# Autodesk Inventor assembly: Лестница
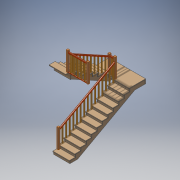
[picture p0: Inventor's stored thumbnail of the model, 180x180]
Saved by Autodesk Inventor 2019 (Build 230136000, 136)
## iProperties
Created: 2018-10-10
Part Number: Лестница
Material: Типовые
Document SubType Name: Assembly
Designer: Андреев Н.Л.
Mass: 392363 g
Surface Area: 432794 cm^2
Volume: 616684 cm^3
Density: 0.636246 g/cm^3
_SolveAssemblyDoc: Frame Generator Solve Assembly
_Version: 15.0.0
Author: Андреев Н.Л.
## Documents named in this file (15)
- C:\Users\andrnl\Documents\Inventor\Мурзин\Лестница.iam
- C:\Users\andrnl\Documents\Inventor\Мурзин\Проступь\Проступь-02.ipt
- C:\Users\andrnl\Documents\Inventor\Мурзин\Проступь.ipt
- C:\Users\andrnl\Documents\Inventor\Мурзин\Марш\Марш-01.iam
- C:\Users\andrnl\Documents\Inventor\Мурзин\Марш.iam
- C:\Users\andrnl\Documents\Inventor\Мурзин\Марш\Марш-02.iam
- C:\Users\andrnl\Documents\Inventor\Мурзин\Столб\Столб-01.ipt
- C:\Users\andrnl\Documents\Inventor\Мурзин\Столб.ipt
- C:\Users\andrnl\Documents\Inventor\Мурзин\Лестница\Frame\Frame0001.iam
- C:\Users\andrnl\Documents\Inventor\Мурзин\Балясина\Балясина-01.ipt
- C:\Users\andrnl\Documents\Inventor\Мурзин\Балясина.ipt
- C:\Users\andrnl\Documents\Inventor\Мурзин\Балясина\Балясина-02.ipt
- C:\Users\andrnl\Documents\Inventor\Мурзин\Проступь\Проступь-01.ipt
- C:\Users\andrnl\Documents\Inventor\Мурзин\Балка.ipt
- C:\Users\andrnl\Documents\Inventor\Мурзин\Лестница Мурзин.xlsx
## Components (42 placed, 9 different names)
1. Проступь-02:1 — Заподлицо:1, Заподлицо:2, Заподлицо:3, Заподлицо:4, Заподлицо:6, Заподлицо:7, Совмещение:1, Совмещение:4, Совмещение:5, Совмещение:7, Заподлицо:13, Заподлицо:17
2. Марш-01:1 [sub-assembly] — Заподлицо:4, Заподлицо:5, Заподлицо:6, Совмещение:2, Заподлицо:9, Совмещение:3, Совмещение:15, Заподлицо:24
3. Марш-02:2 [sub-assembly] — Заподлицо:7, Заподлицо:8, Совмещение:1, Заподлицо:12, Совмещение:6, Совмещение:16, Заподлицо:20, Заподлицо:21, Заподлицо:22
4. Столб-01:1 — Совмещение:2, Заподлицо:9, Совмещение:3, Заподлицо:10, Совмещение:11, Заподлицо:19
5. Столб-01:2 — Заподлицо:10, Заподлицо:11, Совмещение:4, Заподлицо:23, Совмещение:18
6. Столб-01:3 — Совмещение:5, Заподлицо:12, Заподлицо:11, Совмещение:6, Заподлицо:14, Совмещение:13, Совмещение:14
7. Столб-01:4 — Совмещение:7, Заподлицо:13, Заподлицо:14, Заподлицо:15, Заподлицо:16, Совмещение:9, Заподлицо:18
8. Столб-01:5 — Заподлицо:15, Заподлицо:16, Заподлицо:17
9. Frame0001:1 [sub-assembly] — Совмещение:8, Совмещение:10, Совмещение:12, Совмещение:17
10. Проступь-01:2 — Заподлицо:20, Заподлицо:21, Заподлицо:22
11. Балясина-01:28 — Совмещение:17, Заподлицо:23, Совмещение:18
12. Балка:1 — Заподлицо:24
13. Балясина-01:1 — Совмещение:8, Совмещение:9, Заподлицо:18
14. Балясина-01:4
15. Балясина-01:5
16. Балясина-01:6
17. Балясина-01:7
18. Балясина-02:2 — Совмещение:10, Совмещение:11, Заподлицо:19
19. Балясина-02:8
20. Балясина-02:9 — Совмещение:15
21. Балясина-02:10
22. Балясина-02:11
23. Балясина-02:12
24. Балясина-02:13
25. Балясина-02:14
26. Балясина-02:15
27. Балясина-02:16
28. Балясина-02:29
29. Балясина-02:30
30. Балясина-02:31
31. Балясина-02:32
32. Балясина-02:33
33. Балясина-02:3 — Совмещение:12, Совмещение:13, Совмещение:14
34. Балясина-02:17
35. Балясина-02:18 — Совмещение:16
36. Балясина-02:19
37. Балясина-02:20
38. Балясина-02:21
39. Балясина-02:22
40. Балясина-02:23
41. Балясина-02:24
42. Балясина-02:25
## Component patterns: (5 elements, first: Балясина-01:1), (15 elements, first: Балясина-02:2), (10 elements, first: Балясина-02:3)
## Relationships (42: Flush 24, Mate 18)
- Заподлицо:1 [Flush] (5 mm): Проступь-02:1
- Заподлицо:2 [Flush] (5 mm): Проступь-02:1
- Заподлицо:3 [Flush] (-1950 mm): Проступь-02:1
- Заподлицо:4 [Flush]: Проступь-02:1 ↔ Марш-01:1
- Заподлицо:5 [Flush]: Марш-01:1
- Заподлицо:6 [Flush]: Проступь-02:1 ↔ Марш-01:1
- Заподлицо:7 [Flush]: Проступь-02:1 ↔ Марш-02:2
- Заподлицо:8 [Flush]: Марш-02:2
- Совмещение:1 [Mate]: Проступь-02:1 ↔ Марш-02:2
- Совмещение:2 [Mate]: Марш-01:1 ↔ Столб-01:1
- Заподлицо:9 [Flush] (10 mm): Марш-01:1 ↔ Столб-01:1
- Совмещение:3 [Mate]: Марш-01:1 ↔ Столб-01:1
- Заподлицо:10 [Flush]: Столб-01:1 ↔ Столб-01:2
- Заподлицо:11 [Flush]: Столб-01:2 ↔ Столб-01:3
- Совмещение:4 [Mate]: Проступь-02:1 ↔ Столб-01:2
- Совмещение:5 [Mate]: Проступь-02:1 ↔ Столб-01:3
- Заподлицо:12 [Flush] (10 mm): Марш-02:2 ↔ Столб-01:3
- Совмещение:6 [Mate]: Марш-02:2 ↔ Столб-01:3
- Совмещение:7 [Mate] (1300 mm): Проступь-02:1 ↔ Столб-01:4
- Заподлицо:13 [Flush] (3050 mm): Проступь-02:1 ↔ Столб-01:4
- Заподлицо:14 [Flush]: Столб-01:3 ↔ Столб-01:4
- Заподлицо:15 [Flush]: Столб-01:4 ↔ Столб-01:5
- Заподлицо:16 [Flush]: Столб-01:4 ↔ Столб-01:5
- Заподлицо:17 [Flush]: Проступь-02:1 ↔ Столб-01:5
- Совмещение:8 [Mate]: Frame0001:1 ↔ Балясина-01:1
- Совмещение:9 [Mate] (150 mm): Столб-01:4 ↔ Балясина-01:1
- Заподлицо:18 [Flush]: Столб-01:4 ↔ Балясина-01:1
- Совмещение:10 [Mate]: Frame0001:1 ↔ Балясина-02:2
- Совмещение:11 [Mate] (150 mm): Столб-01:1 ↔ Балясина-02:2
- Заподлицо:19 [Flush]: Столб-01:1 ↔ Балясина-02:2
- Совмещение:12 [Mate]: Frame0001:1 ↔ Балясина-02:3
- Совмещение:13 [Mate] (150 mm): Столб-01:3 ↔ Балясина-02:3
- Совмещение:14 [Mate]: Столб-01:3 ↔ Балясина-02:3
- Совмещение:15 [Mate]: Марш-01:1 ↔ Балясина-02:9
- Совмещение:16 [Mate]: Марш-02:2 ↔ Балясина-02:18
- Заподлицо:20 [Flush]: Марш-02:2 ↔ Проступь-01:2
- Заподлицо:21 [Flush] (-162.5 mm): Марш-02:2 ↔ Проступь-01:2
- Заподлицо:22 [Flush] (296.8 mm): Марш-02:2 ↔ Проступь-01:2
- Совмещение:17 [Mate]: Frame0001:1 ↔ Балясина-01:28
- Заподлицо:23 [Flush]: Столб-01:2 ↔ Балясина-01:28
- Совмещение:18 [Mate] (80 mm): Столб-01:2 ↔ Балясина-01:28
- Заподлицо:24 [Flush]: Марш-01:1 ↔ Балка:1
## Named parameters: зУр2Эт = 3250 mm, зДл = 3000 mm, зШир = 2000 mm, пДлПроступи = 900 mm, пПодъемов = 20, пПодъем = 162.5 mm, пХод = 296.8 mm, пЭффШаг = 621.8 mm, пСвес = 30.2 mm, пТолПроступи = 40 mm, пТолКосоура = 40 mm, пТолСтолба = 90 mm, пТолБалясины = 40 mm, пШирКосоура = 300 mm, пОтступСтен = 5 mm, пДиаг = 338.3733 mm, пПлощадка = 1, пПодъемов2 = 7, пВыход2Ур = 1, пПодъемов1 = 11, пШирПроступи = 327 mm, пТолПодступенка = 17.4 mm, пШипПодступ = 10 mm, пОтступШипа = 50 mm, пГлубПаза = 12 mm, пОтступПодступ = 10 mm, пОтступОтСтен = 5 mm, пДлПлощадки = 1990 mm, пТолПричала = 17.4 mm, зТолПерекрытия = 300 mm, пСвесВбок = 30 mm, Балюстрада = 150 mm
